# Autodesk Inventor assembly: systèmeMoteur6G
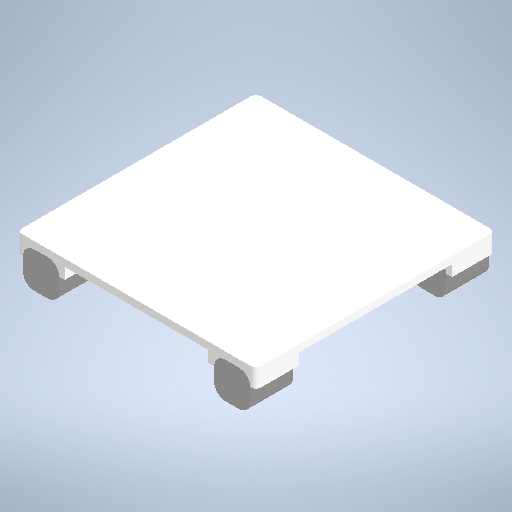
[picture p0: Inventor's stored thumbnail of the model, 512x512]
Saved by Autodesk Inventor 2025.2 (Build 292293000, 293)
## iProperties
Created: 2025-02-21
Part Number: systèmeMoteur6G
Document SubType Name: Assembly
Designer: antoi
Author: antoi
## Documents named in this file (3)
- C:\Users\antoi\Documents\Henallux_24_25\Q2\proj\prototype\systèmeMoteur6G.iam
- C:\Users\antoi\Documents\Henallux_24_25\Q2\proj\prototype\plateauMoteur6G.ipt
- C:\Users\antoi\Documents\Henallux_24_25\Q2\proj\prototype\Moteur6G.ipt
## Components (5 placed, 2 different names)
1. plateauMoteur6G:1 — Placage:1, Placage:2, Affleurement:1
2. Moteur6G:1 — Placage:1, Placage:2, Affleurement:1
3. Moteur6G:2
4. Moteur6G:3
5. Moteur6G:4
## Component patterns: (4 elements, first: Moteur6G:1)
## Relationships (3: Mate 2, Flush 1)
- Placage:1 [Mate]: plateauMoteur6G:1 ↔ Moteur6G:1
- Placage:2 [Mate]: plateauMoteur6G:1 ↔ Moteur6G:1
- Affleurement:1 [Flush]: plateauMoteur6G:1 ↔ Moteur6G:1
